# Autodesk Inventor assembly: Dispensador
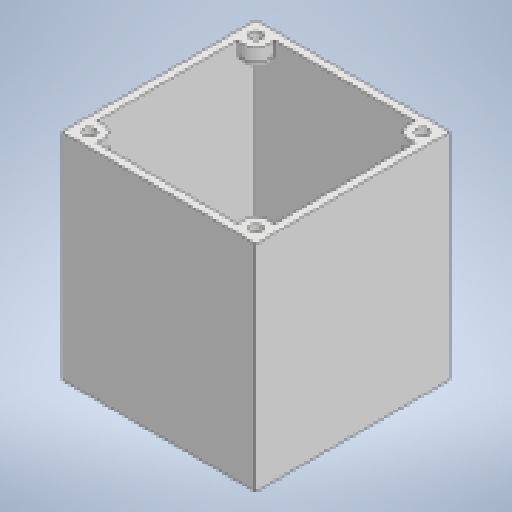
[picture p0: Inventor's stored thumbnail of the model, 512x512]
Saved by Autodesk Inventor 2024 (Build 280153000, 153)
## iProperties
Created: 2025-03-02
Part Number: Dispensador
Document SubType Name: Assembly
Designer: sergi
Author: sergi
## Documents named in this file (4)
- C:\Users\sergi\OneDrive\Escritorio\Projects\16. Protection catapult\Inventor\Dispensador.iam
- C:\Users\sergi\OneDrive\Escritorio\Projects\16. Protection catapult\Inventor\Base dispensador.ipt
- C:\Users\sergi\OneDrive\Escritorio\Projects\16. Protection catapult\Inventor\Tapa dispensador.ipt
- C:\Users\sergi\OneDrive\Escritorio\Projects\16. Protection catapult\Inventor\Parte deslizante.ipt
## Components (3 placed, 3 different names)
1. Base dispensador:1 — Nivelación:1, Coincidencia:1, Coincidencia:2, Coincidencia:3
2. Tapa dispensador:1 — Nivelación:1
3. Parte deslizante:1 — Coincidencia:1, Coincidencia:2, Coincidencia:3
## Relationships (4: Mate 3, Flush 1)
- Nivelación:1 [Flush]: Base dispensador:1 ↔ Tapa dispensador:1
- Coincidencia:1 [Mate] (4 mm): Base dispensador:1 ↔ Parte deslizante:1
- Coincidencia:2 [Mate] (1.5 mm): Base dispensador:1 ↔ Parte deslizante:1
- Coincidencia:3 [Mate] (1.5 mm): Base dispensador:1 ↔ Parte deslizante:1
